# Autodesk Inventor assembly: coffeetable
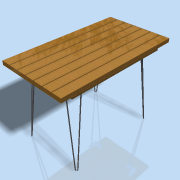
[picture p0: Inventor's stored thumbnail of the model, 180x180]
Saved by Autodesk Inventor 2019 (Build 230136000, 136)
## iProperties
Created: 2019-12-05
Part Number: coffeetable
Document SubType Name: Assembly
Designer: qitilab4
Author: qitilab4
## Documents named in this file (4)
- C:\Users\qitilab4\Documents\coffeetable\coffeetable.iam
- C:\Users\qitilab4\Documents\coffeetable\2x4.ipt
- C:\Users\qitilab4\Documents\coffeetable\plywood.ipt
- C:\Users\qitilab4\Documents\coffeetable\hair pin leg.ipt
## Components (12 placed, 3 different names)
1. plywood:1 — Mate:1, Flush:1, Flush:2, Mate:5, Flush:9, Flush:10
2. hair pin leg:1 — Mate:3, Flush:4, Flush:5, Flush:8, Mate:4
3. hair pin leg:2 — Flush:5, Flush:7, Flush:8, Mate:4
4. hair pin leg:3 — Mate:2, Flush:3, Flush:6, Flush:7, Flush:9, Flush:10
5. hair pin leg:4 — Mate:2, Flush:3, Mate:3, Flush:4, Flush:6, Mate:5
6. 2x4:1
7. 2x4:2
8. 2x4:3
9. 2x4:4
10. 2x4:5
11. 2x4:6
12. 2x4:7 — Mate:1, Flush:1, Flush:2
## Component patterns: (7 elements, first: 2x4:1)
## Relationships (15: Flush 10, Mate 5)
- Mate:1: plywood:1 ↔ 2x4:7
- Flush:1 (-10.795 mm): plywood:1 ↔ 2x4:7
- Flush:2 (-133.35 mm): plywood:1 ↔ 2x4:7
- Mate:2 (-558.8 mm): hair pin leg:3 ↔ hair pin leg:4
- Flush:3: hair pin leg:3 ↔ hair pin leg:4
- Mate:3 (-863.6 mm): hair pin leg:1 ↔ hair pin leg:4
- Flush:4: hair pin leg:1 ↔ hair pin leg:4
- Flush:5: hair pin leg:1 ↔ hair pin leg:2
- Flush:6: hair pin leg:3 ↔ hair pin leg:4
- Flush:7: hair pin leg:2 ↔ hair pin leg:3
- Flush:8: hair pin leg:1 ↔ hair pin leg:2
- Mate:4 (-609.6 mm): hair pin leg:1 ↔ hair pin leg:2
- Mate:5: plywood:1 ↔ hair pin leg:4
- Flush:9 (25.4 mm): plywood:1 ↔ hair pin leg:3
- Flush:10 (25.4 mm): plywood:1 ↔ hair pin leg:3
